# Autodesk Inventor assembly: Balancer
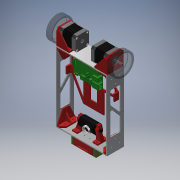
[picture p0: Inventor's stored thumbnail of the model, 180x180]
Saved by Autodesk Inventor 2018 (Build 220112000, 112)
## iProperties
Part Number: Balancer
Material: Ogólny
Document SubType Name: Assembly
Designer: Wojciech
Mass: 558.3 g
Surface Area: 2091.19 cm^2
Volume: 525.938 cm^3
Density: 1.06153 g/cm^3
Author: Wojciech
## Documents named in this file (13)
- C:\Users\Wojciech\Documents\Projekty\Balancer\Model 3D\Balancer.iam
- C:\Users\Wojciech\Documents\Projekty\Balancer\Model 3D\Koło.ipt
- C:\Users\Wojciech\Documents\Projekty\Balancer\Model 3D\Silnik_Obudowa.ipt
- C:\Users\Wojciech\Documents\Projekty\Balancer\Model 3D\Podstawa.ipt
- C:\Users\Wojciech\Documents\Projekty\Balancer\Model 3D\Wspornik.ipt
- C:\Users\Wojciech\Documents\Projekty\Balancer\Model 3D\Bok.ipt
- C:\Users\Wojciech\Documents\Projekty\Balancer\Model 3D\Góra.ipt
- C:\Users\Wojciech\Documents\Projekty\Balancer\Model 3D\Kamera_w_uchwycie.ipt
- C:\Users\Wojciech\Documents\Projekty\Balancer\Model 3D\Wspornik_góra.ipt
- C:\Users\Wojciech\Documents\Projekty\Balancer\Model 3D\Li-Pol_uchwyt.ipt
- C:\Users\Wojciech\Documents\Projekty\Balancer\Model 3D\Li-Pol.ipt
- C:\Users\Wojciech\Documents\Projekty\Balancer\Model 3D\RPI.ipt
- C:\Users\Wojciech\Documents\Projekty\Balancer\Model 3D\Uchwyt_elektronika.ipt
## Components (17 placed, 12 different names)
1. Silnik_Obudowa:1 — Zestawiający:4, Zestawiający:5, Zestawiający:6, Zestawiający:7, Zestawiający:10
2. Silnik_Obudowa:2 — Zestawiający:1, Zestawiający:2, Zestawiający:3, Zestawiający:8, Zestawiający:9
3. Podstawa:1 — Zestawiający:1, Zestawiający:2, Zestawiający:3, Zestawiający:4, Zestawiający:5, Zestawiający:6, Zestawiający:11, Zestawiający:12, Zestawiający:13, Zestawiający:14, Zestawiający:15, Zestawiający:16, Zestawiający:17, Równoległy:1, Zestawiający:20, Równoległy:2, Zestawiający:37
4. Koło:1 — Zestawiający:7, Zestawiający:10
5. Koło:2 — Zestawiający:8, Zestawiający:9
6. Wspornik:1 — Zestawiający:11, Zestawiający:12, Zestawiający:13, Zestawiający:18, Zestawiający:19
7. Wspornik:2 — Zestawiający:14, Zestawiający:15, Zestawiający:16, Zestawiający:21, Zestawiający:22
8. Bok:1 — Zestawiający:17, Równoległy:1, Zestawiający:18, Zestawiający:19, Równoległy:3, Zestawiający:23, Równoległy:4, Zestawiający:29, Równoległy:6, Zestawiający:38
9. Bok:2 — Zestawiający:20, Zestawiający:21, Równoległy:2, Zestawiający:22, Zestawiający:28, Równoległy:5, Zestawiający:39
10. Góra:1 — Równoległy:3, Zestawiający:23, Równoległy:4, Zestawiający:24, Zestawiający:25, Zestawiający:26, Zestawiający:27, Zestawiający:30, Zestawiający:31, Zestawiający:32, Zestawiający:33
11. Kamera_w_uchwycie:1 — Zestawiający:24, Zestawiający:25, Zestawiający:26
12. Wspornik_góra:1 — Zestawiający:27, Zestawiający:28, Równoległy:5
13. Wspornik_góra:2 — Zestawiający:29, Zestawiający:30, Równoległy:6
14. Li-Pol_uchwyt:1 — Zestawiający:31, Zestawiający:32, Zestawiający:33, Zestawiający:34, Zestawiający:35, Równoległy:7
15. Li-Pol:1 — Zestawiający:34, Zestawiający:35, Równoległy:7
16. RPI:1 — Zestawiający:40, Zestawiający:41
17. Uchwyt_elektronika:1 — Zestawiający:37, Zestawiający:38, Zestawiający:39, Zestawiający:40, Zestawiający:41
## Relationships (47: Mate 40, Flush 7)
- Zestawiający:1 [Mate]: Silnik_Obudowa:2 ↔ Podstawa:1
- Zestawiający:2 [Mate]: Silnik_Obudowa:2 ↔ Podstawa:1
- Zestawiający:3 [Mate]: Silnik_Obudowa:2 ↔ Podstawa:1
- Zestawiający:4 [Mate]: Silnik_Obudowa:1 ↔ Podstawa:1
- Zestawiający:5 [Mate]: Silnik_Obudowa:1 ↔ Podstawa:1
- Zestawiający:6 [Mate]: Silnik_Obudowa:1 ↔ Podstawa:1
- Zestawiający:7 [Mate]: Silnik_Obudowa:1 ↔ Koło:1
- Zestawiający:8 [Mate]: Silnik_Obudowa:2 ↔ Koło:2
- Zestawiający:9 [Mate]: Silnik_Obudowa:2 ↔ Koło:2
- Zestawiający:10 [Mate]: Silnik_Obudowa:1 ↔ Koło:1
- Zestawiający:11 [Mate]: Podstawa:1 ↔ Wspornik:1
- Zestawiający:12 [Mate]: Podstawa:1 ↔ Wspornik:1
- Zestawiający:13 [Mate]: Podstawa:1 ↔ Wspornik:1
- Zestawiający:14 [Mate]: Podstawa:1 ↔ Wspornik:2
- Zestawiający:15 [Mate]: Podstawa:1 ↔ Wspornik:2
- Zestawiający:16 [Mate]: Podstawa:1 ↔ Wspornik:2
- Zestawiający:17 [Mate]: Podstawa:1 ↔ Bok:1
- Równoległy:1 [Flush]: Podstawa:1 ↔ Bok:1
- Zestawiający:18 [Mate]: Wspornik:1 ↔ Bok:1
- Zestawiający:19 [Mate]: Wspornik:1 ↔ Bok:1
- Zestawiający:20 [Mate]: Podstawa:1 ↔ Bok:2
- Zestawiający:21 [Mate]: Wspornik:2 ↔ Bok:2
- Równoległy:2 [Flush]: Podstawa:1 ↔ Bok:2
- Zestawiający:22 [Mate]: Wspornik:2 ↔ Bok:2
- Równoległy:3 [Flush]: Bok:1 ↔ Góra:1
- Zestawiający:23 [Mate]: Bok:1 ↔ Góra:1
- Równoległy:4 [Flush]: Bok:1 ↔ Góra:1
- Zestawiający:24 [Mate]: Góra:1 ↔ Kamera_w_uchwycie:1
- Zestawiający:25 [Mate]: Góra:1 ↔ Kamera_w_uchwycie:1
- Zestawiający:26 [Mate]: Góra:1 ↔ Kamera_w_uchwycie:1
- Zestawiający:27 [Mate]: Góra:1 ↔ Wspornik_góra:1
- Zestawiający:28 [Mate]: Bok:2 ↔ Wspornik_góra:1
- Równoległy:5 [Flush]: Bok:2 ↔ Wspornik_góra:1
- Zestawiający:29 [Mate]: Bok:1 ↔ Wspornik_góra:2
- Zestawiający:30 [Mate]: Góra:1 ↔ Wspornik_góra:2
- Równoległy:6 [Flush]: Bok:1 ↔ Wspornik_góra:2
- Zestawiający:31 [Mate]: Góra:1 ↔ Li-Pol_uchwyt:1
- Zestawiający:32 [Mate]: Góra:1 ↔ Li-Pol_uchwyt:1
- Zestawiający:33 [Mate]: Góra:1 ↔ Li-Pol_uchwyt:1
- Zestawiający:34 [Mate]: Li-Pol_uchwyt:1 ↔ Li-Pol:1
- Zestawiający:35 [Mate]: Li-Pol_uchwyt:1 ↔ Li-Pol:1
- Równoległy:7 [Flush] (-8.5 mm): Li-Pol_uchwyt:1 ↔ Li-Pol:1
- Zestawiający:37 [Mate]: Podstawa:1 ↔ Uchwyt_elektronika:1
- Zestawiający:38 [Mate]: Bok:1 ↔ Uchwyt_elektronika:1
- Zestawiający:39 [Mate]: Bok:2 ↔ Uchwyt_elektronika:1
- Zestawiający:40 [Mate]: RPI:1 ↔ Uchwyt_elektronika:1
- Zestawiający:41 [Mate]: RPI:1 ↔ Uchwyt_elektronika:1
